# Autodesk Inventor assembly: Assembly1
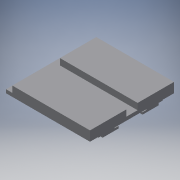
[picture p0: Inventor's stored thumbnail of the model, 180x180]
Saved by Autodesk Inventor 2019 (Build 230136000, 136)
## iProperties
Created: 2018-12-29
Part Number: Assembly1
Document SubType Name: Assembly
Designer: Owner
Author: Owner
## Documents named in this file (4)
- D:\Galx_1133 Selector 6 box\Assembly1.iam
- D:\Galx_1133 Selector 6 box\Part_A.ipt
- D:\Galx_1133 Selector 6 box\Part_B.ipt
- D:\Galx_1133 Selector 6 box\Part_C.ipt
## Components (7 placed, 3 different names)
1. Part_A:1 — Mate:2, Flush:3, Flush:4
2. Part_A:2 — Mate:1, Flush:1, Flush:2
3. Part_B:1 — Mate:1, Flush:1, Flush:2, Mate:2, Flush:3, Flush:4, Mate:3, Flush:5, Flush:6, Mate:4, Flush:7, Flush:8
4. Part_C:1 — Mate:3, Flush:5, Flush:6, Mate:6, Flush:11, Flush:12
5. Part_C:2 — Mate:6, Flush:11, Flush:12
6. Part_C:3 — Mate:5, Flush:9, Flush:10
7. Part_C:4 — Mate:4, Flush:7, Flush:8, Mate:5, Flush:9, Flush:10
## Relationships (18: Flush 12, Mate 6)
- Mate:1: Part_A:2 ↔ Part_B:1
- Flush:1: Part_A:2 ↔ Part_B:1
- Flush:2: Part_A:2 ↔ Part_B:1
- Mate:2: Part_A:1 ↔ Part_B:1
- Flush:3: Part_A:1 ↔ Part_B:1
- Flush:4: Part_A:1 ↔ Part_B:1
- Mate:3: Part_B:1 ↔ Part_C:1
- Flush:5: Part_B:1 ↔ Part_C:1
- Flush:6 (22.225 mm): Part_B:1 ↔ Part_C:1
- Mate:4: Part_B:1 ↔ Part_C:4
- Flush:7 (-22.225 mm): Part_B:1 ↔ Part_C:4
- Flush:8: Part_B:1 ↔ Part_C:4
- Mate:5: Part_C:3 ↔ Part_C:4
- Flush:9: Part_C:3 ↔ Part_C:4
- Flush:10 (9.525 mm): Part_C:3 ↔ Part_C:4
- Mate:6: Part_C:1 ↔ Part_C:2
- Flush:11: Part_C:1 ↔ Part_C:2
- Flush:12 (9.525 mm): Part_C:1 ↔ Part_C:2
